# Autodesk Inventor assembly: V Wheel and Bearings
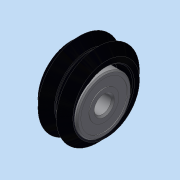
[picture p0: Inventor's stored thumbnail of the model, 180x180]
Saved by Autodesk Inventor 2013 (Build 170138000, 138)
## iProperties
Created: 2013-06-21
Part Number: V Wheel and Bearings
Document SubType Name: Assembly
Designer: Jon Hollander
Author: Jon Hollander
## Documents named in this file (4)
- D:\Dropbox\Research\CAD Library\v-slot\V Wheel and Bearings.iam
- D:\Dropbox\Research\CAD Library\v-slot\Dual V Wheel.ipt
- D:\Dropbox\Research\CAD Library\v-slot\Part Assemblies\Idler Pulley - Spacer - Bolt\Libraries\Content Center Files\en-US\5mm Precision Washer\5mm Precision Washer.ipt
- D:\Dropbox\Research\CAD Library\v-slot\Bearing - 625 2RS\625 2RS Bearing.ipt
## Components (4 placed, 3 different names)
1. Dual V Wheel:1 — Mate:5, Mate:6
2. 625 2RS Bearing:1 — Mate:1, Mate:2, Mate:3
3. 625 2RS Bearing:2 — Mate:3, Mate:4, Mate:5
4. 5mm Precision Washer 5mm Precision Washer:1 — Mate:1, Mate:2, Mate:4, Mate:6
## Relationships (6: Mate 6)
- Mate:1: 625 2RS Bearing:1 ↔ 5mm Precision Washer 5mm Precision Washer:1
- Mate:2: 625 2RS Bearing:1 ↔ 5mm Precision Washer 5mm Precision Washer:1
- Mate:3: 625 2RS Bearing:1 ↔ 625 2RS Bearing:2
- Mate:4: 625 2RS Bearing:2 ↔ 5mm Precision Washer 5mm Precision Washer:1
- Mate:5: Dual V Wheel:1 ↔ 625 2RS Bearing:2
- Mate:6 (0.6 mm): Dual V Wheel:1 ↔ 5mm Precision Washer 5mm Precision Washer:1
